# Autodesk Inventor assembly: Assembly
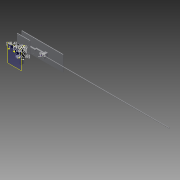
[picture p0: Inventor's stored thumbnail of the model, 180x180]
Saved by Autodesk Inventor 2014 SP1 (Build 180222100, 222)
## iProperties
Created: 2014-02-07
Part Number: Assembly
Document SubType Name: Assembly
Designer: Owner
Author: Owner
## Documents named in this file (11)
- C:\Users\Owner\Documents\GitHub\Team2083-2014-CAD\Winebago Concept\Generation 2\Assembly.iam
- C:\Users\Owner\Documents\GitHub\Team2083-2014-CAD\Winebago Concept\Generation 2\big plate.ipt
- C:\Users\Owner\Documents\GitHub\Team2083-2014-CAD\Winebago Concept\Generation 2\small plate.ipt
- C:\Users\Owner\Documents\GitHub\Team2083-2014-CAD\Winebago Concept\Window Motor\ND Motor Right.ipt
- C:\Users\Owner\Documents\GitHub\Team2083-2014-CAD\Winebago Concept\Generation 2\motor connector.ipt
- C:\Users\Owner\Documents\GitHub\Team2083-2014-CAD\Winebago Concept\3 in bar.ipt
- C:\Users\Owner\Documents\GitHub\Team2083-2014-CAD\Winebago Concept\1 in rod.ipt
- C:\Users\Owner\Documents\GitHub\Team2083-2014-CAD\Winebago Concept\5 in bar.ipt
- C:\Users\Owner\Documents\GitHub\Team2083-2014-CAD\Winebago Concept\right angle rod holder.ipt
- C:\Users\Owner\Documents\GitHub\Team2083-2014-CAD\Winebago Concept\50 in rod.ipt
- C:\Users\Owner\Documents\GitHub\Team2083-2014-CAD\Winebago Concept\Generation 2\rod guide.ipt
## Components (13 placed, 10 different names)
1. big plate:1 — Mate:1, Mate:2, Mate:3, Mate:4, Mate:10, Mate:11, Mate:12
2. small plate:1 — Mate:1, Mate:2, Mate:3, Mate:4, Mate:5, Mate:6, Mate:7, Flush:1
3. ND Motor Right:1 — Mate:5, Mate:6, Mate:7, Mate:8, Mate:9
4. motor connector:1 — Mate:8, Mate:9, Flush:1, Insert:1
5. 3 in bar:1 — Insert:1, Insert:2, Insert:3
6. 1 in rod:1 — Insert:5, Insert:6
7. 1 in rod:2 — Insert:3, Insert:4
8. 1 in rod:3 — Insert:2
9. 5 in bar:1 — Insert:4, Insert:5
10. 5 in bar:2 — Insert:6, Insert:7
11. right angle rod holder:1 — Insert:7, Insert:8
12. 50 in rod:1 — Insert:8, Mate:13
13. rod guide:1 — Mate:10, Mate:11, Mate:12, Mate:13
## Relationships (22: Mate 13, Insert 8, Flush 1)
- Mate:1: big plate:1 ↔ small plate:1
- Mate:2: big plate:1 ↔ small plate:1
- Mate:3: big plate:1 ↔ small plate:1
- Mate:4 (38.1 mm): big plate:1 ↔ small plate:1
- Mate:5: small plate:1 ↔ ND Motor Right:1
- Mate:6: small plate:1 ↔ ND Motor Right:1
- Mate:7: small plate:1 ↔ ND Motor Right:1
- Mate:8: ND Motor Right:1 ↔ motor connector:1
- Mate:9 (2.54 mm): ND Motor Right:1 ↔ motor connector:1
- Flush:1 (-12.7 mm): small plate:1 ↔ motor connector:1
- Insert:1: motor connector:1 ↔ 3 in bar:1
- Insert:2: 3 in bar:1 ↔ 1 in rod:3
- Insert:3: 3 in bar:1 ↔ 1 in rod:2
- Insert:4: 1 in rod:2 ↔ 5 in bar:1
- Insert:5: 1 in rod:1 ↔ 5 in bar:1
- Insert:6: 1 in rod:1 ↔ 5 in bar:2
- Insert:7: 5 in bar:2 ↔ right angle rod holder:1
- Insert:8: right angle rod holder:1 ↔ 50 in rod:1
- Mate:10: big plate:1 ↔ rod guide:1
- Mate:11: big plate:1 ↔ rod guide:1
- Mate:12: big plate:1 ↔ rod guide:1
- Mate:13: 50 in rod:1 ↔ rod guide:1
